# Autodesk Inventor assembly: Assembly1
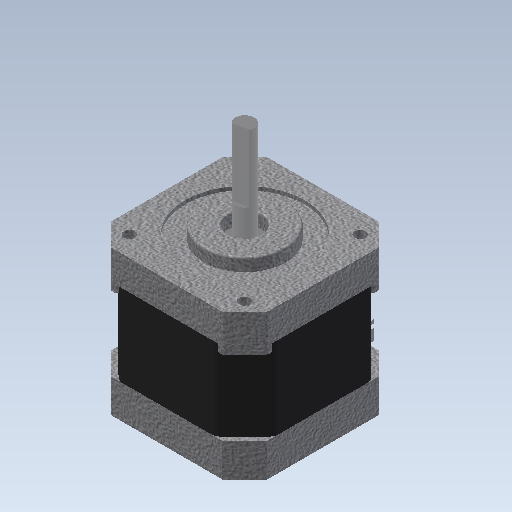
[picture p0: Inventor's stored thumbnail of the model, 512x512]
Saved by Autodesk Inventor 2021 (Build 250183000, 183)
## iProperties
Created: 2020-07-01
Part Number: Assembly1
Document SubType Name: Assembly
Designer: IVAN
Author: IVAN
## Documents named in this file (7)
- C:\Users\ASUS\Downloads\stepper-motor-nema17-17hs4401-42-mm-1.snapshot.1\Assembly1.iam
- C:\Users\ASUS\Downloads\stepper-motor-nema17-17hs4401-42-mm-1.snapshot.1\Part1.ipt
- C:\Users\ASUS\Downloads\stepper-motor-nema17-17hs4401-42-mm-1.snapshot.1\Part2.ipt
- C:\Users\ASUS\Downloads\stepper-motor-nema17-17hs4401-42-mm-1.snapshot.1\Part4.ipt
- C:\Users\ASUS\Downloads\stepper-motor-nema17-17hs4401-42-mm-1.snapshot.1\Part5.ipt
- C:\Users\ASUS\Downloads\stepper-motor-nema17-17hs4401-42-mm-1.snapshot.1\Part6.ipt
- C:\Users\ASUS\Downloads\stepper-motor-nema17-17hs4401-42-mm-1.snapshot.1\Part7.ipt
## Components (9 placed, 6 different names)
1. Part1:1 — Mate:1, Flush:1, Flush:2, Mate:4, Flush:6, Flush:7, Mate:5, Mate:6, Mate:7, Mate:8, Mate:9, Mate:10, Mate:11, Mate:12
2. Part2:1 — Mate:1, Flush:1, Flush:2, Mate:2, Flush:3, Flush:4
3. Part4:1 — Mate:2, Flush:3, Flush:4, Mate:3, Flush:5
4. Part5:1 — Mate:3, Flush:5
5. Part6:1 — Mate:4, Flush:6, Flush:7
6. Part7:1 — Mate:5, Mate:6
7. Part7:2 — Mate:7, Mate:8
8. Part7:3 — Mate:9, Mate:10
9. Part7:4 — Mate:11, Mate:12
## Relationships (19: Mate 12, Flush 7)
- Mate:1: Part1:1 ↔ Part2:1
- Flush:1: Part1:1 ↔ Part2:1
- Flush:2: Part1:1 ↔ Part2:1
- Mate:2: Part2:1 ↔ Part4:1
- Flush:3: Part2:1 ↔ Part4:1
- Flush:4: Part2:1 ↔ Part4:1
- Mate:3: Part4:1 ↔ Part5:1
- Flush:5 (-23.5 mm): Part4:1 ↔ Part5:1
- Mate:4: Part1:1 ↔ Part6:1
- Flush:6 (-1 mm): Part1:1 ↔ Part6:1
- Flush:7 (0.25 mm): Part1:1 ↔ Part6:1
- Mate:5: Part1:1 ↔ Part7:1
- Mate:6: Part1:1 ↔ Part7:1
- Mate:7: Part1:1 ↔ Part7:2
- Mate:8: Part1:1 ↔ Part7:2
- Mate:9: Part1:1 ↔ Part7:3
- Mate:10: Part1:1 ↔ Part7:3
- Mate:11: Part1:1 ↔ Part7:4
- Mate:12: Part1:1 ↔ Part7:4
